# Autodesk Inventor assembly: Ensamblaje Lampara
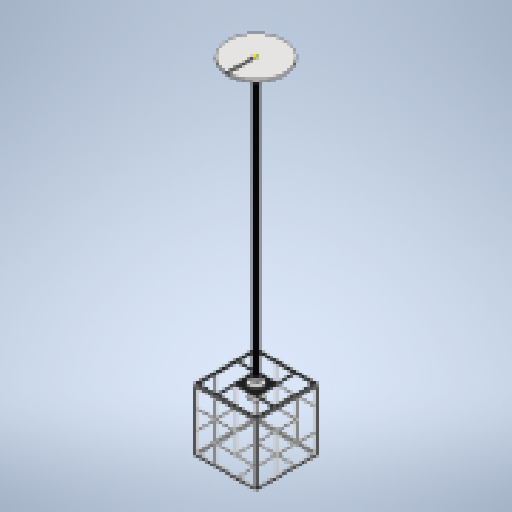
[picture p0: Inventor's stored thumbnail of the model, 512x512]
Saved by Autodesk Inventor 2024 (Build 280153000, 153)
## iProperties
Created: 2024-04-05
Part Number: Ensamblaje Lampara
Document SubType Name: Assembly
Designer: sergi
Author: sergi
## Documents named in this file (5)
- C:\Users\sergi\OneDrive\Escritorio\proyectos\Salon Piso Laguna\Ensamblaje Lampara.iam
- C:\Users\sergi\OneDrive\Escritorio\proyectos\LamparaSalon\Barra.ipt
- C:\Users\sergi\OneDrive\Escritorio\proyectos\LamparaSalon\Processed_Acople E27.ipt
- C:\Users\sergi\OneDrive\Escritorio\proyectos\LamparaSalon\Pie2.ipt
- C:\Users\sergi\OneDrive\Escritorio\proyectos\LamparaSalon\EnsamblajeLampara.iam
## Components (4 placed, 4 different names)
1. Barra:1
2. Processed_Acople E27:1
3. Pie2:1
4. EnsamblajeLampara:1 [sub-assembly]
## Relationships (6: Mate 4, Flush 2)
- [Mate]: Barra:1 ↔ Processed_Acople E27:1
- [Flush]: Barra:1 ↔ Processed_Acople E27:1
- [Mate]: Barra:1 ↔ EnsamblajeLampara:1
- [Flush]: Barra:1 ↔ EnsamblajeLampara:1
- [Mate]: Barra:1 ↔ Pie2:1
- [Mate]: Barra:1 ↔ Pie2:1
## Named parameters: d40_d4 = 0 mm, d41_d5 = 0 mm, d42_d38 = 0 mm, d43_d39 = 0 mm
